# Autodesk Inventor assembly: block_befetigung
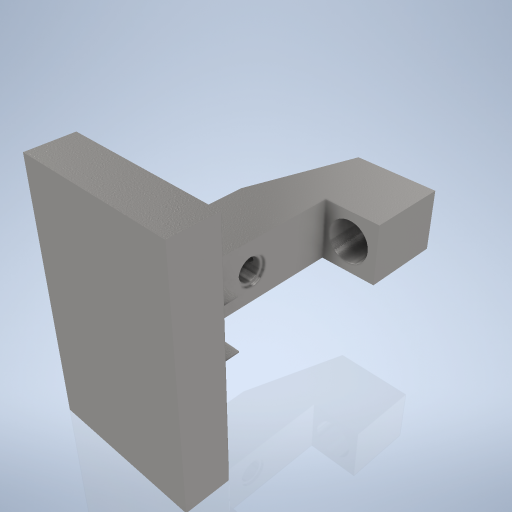
[picture p0: Inventor's stored thumbnail of the model, 512x512]
Saved by Autodesk Inventor 2024.2 (Build 282272000, 272)
## iProperties
Created: 2024-04-30
Part Number: block_befetigung
Document SubType Name: Assembly
Designer: Fabri
Author: Fabri
## Documents named in this file (4)
- C:\Users\Fabri\Documents\Inventor\Motor\block_befetigung.iam
- C:\Users\Fabri\Documents\Inventor\Motor\Grundplatte.ipt
- C:\Users\Fabri\Documents\Inventor\Motor\Bügelbefestigung.ipt
- C:\Users\Fabri\Documents\Inventor\Motor\MotorBlock.ipt
## Components (3 placed, 3 different names)
1. Grundplatte:1 — Einfügen:1
2. Bügelbefestigung:1 — Einfügen:1, Einfügen:2
3. MotorBlock:1 — Einfügen:2
## Relationships (2: Insert 2)
- Einfügen:1 [Insert]: Grundplatte:1 ↔ Bügelbefestigung:1
- Einfügen:2 [Insert]: Bügelbefestigung:1 ↔ MotorBlock:1
